# Autodesk Inventor assembly: Caster
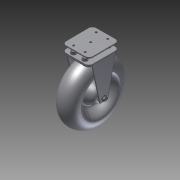
[picture p0: Inventor's stored thumbnail of the model, 180x180]
Saved by Autodesk Inventor 2012 (Build 160160000, 160)
## iProperties
Created: 2011-10-20
Part Number: Caster
Document SubType Name: Assembly
Designer: robotics
Author: robotics
## Documents named in this file (11)
- C:\Users\Tushar\Dropbox\CAD Inventor\Preseason Projects\Cart Competition Cart\Team 2374\Caster.iam
- C:\Users\Tushar\Dropbox\CAD Inventor\Preseason Projects\Cart Competition Cart\Team 2374\Caster2.ipt
- C:\Users\Tushar\Dropbox\CAD Inventor\Preseason Projects\Cart Competition Cart\Team 2374\Wheel.ipt
- C:\Users\Tushar\Dropbox\CAD Inventor\Preseason Projects\Cart Competition Cart\Team 2374\Spacer - .5 x .25.ipt
- C:\Users\Tushar\Dropbox\CAD Inventor\Preseason Projects\Cart Competition Cart\Team 2374\Caster\Design Accelerator\Bolted Connection1.iam
- C:\Users\Tushar\Dropbox\CAD Inventor\Preseason Projects\Cart Competition Cart\Team 2374\Rotation Base.ipt
- C:\Users\Tushar\Dropbox\CAD Inventor\Preseason Projects\Cart Competition Cart\Team 2374\Rotation Top.ipt
- C:\Users\Tushar\Dropbox\CAD Inventor\Preseason Projects\Cart Competition Cart\Team 2374\Caster\Design Accelerator\Bolted Connection2.iam
- C:\Users\Tushar\Dropbox\CAD Inventor\Preseason Projects\Cart Competition Cart\Team 2374\Caster\Design Accelerator\Bolted Connection3.iam
- C:\Users\Tushar\Dropbox\CAD Inventor\Preseason Projects\Cart Competition Cart\Team 2374\Caster\Design Accelerator\Bolted Connection4.iam
- C:\Users\Tushar\Dropbox\CAD Inventor\Preseason Projects\Cart Competition Cart\Team 2374\Caster\Design Accelerator\Bolted Connection5.iam
## Components (11 placed, 6 different names)
1. Caster2:1 — Mate:1, Mate:2, Mate:3, Mate:4, Mate:5, Mate:6, Mate:7, Flush:1, Mate:12, Flush:2, Mate:23, Mate:24
2. Wheel:1 — Mate:1, Mate:2, Mate:3
3. Spacer - .5 x .25:1 — Mate:4, Mate:5
4. Spacer - .5 x .25:2 — Mate:6, Mate:7
5. Bolted Connection:1 [sub-assembly] — Mate:23, Mate:24
6. Rotation Base:1 — Mate:10, Mate:11, Flush:1, Mate:12, Flush:2, Mate:13, Mate:14, Mate:15, Mate:16, Mate:17, Mate:18, Mate:19, Mate:20
7. Rotation Top:1 — Mate:10, Mate:11
8. Bolted Connection:2 [sub-assembly] — Mate:13, Mate:14
9. Bolted Connection:3 [sub-assembly] — Mate:15, Mate:16
10. Bolted Connection:4 [sub-assembly] — Mate:17, Mate:18
11. Bolted Connection:5 [sub-assembly] — Mate:19, Mate:20
## Relationships (22: Mate 20, Flush 2)
- Mate:1 (6.35 mm): Caster2:1 ↔ Wheel:1
- Mate:2 (111.125 mm): Caster2:1 ↔ Wheel:1
- Mate:3 (-50.8 mm): Caster2:1 ↔ Wheel:1
- Mate:4: Caster2:1 ↔ Spacer - .5 x .25:1
- Mate:5: Caster2:1 ↔ Spacer - .5 x .25:1
- Mate:6: Caster2:1 ↔ Spacer - .5 x .25:2
- Mate:7: Caster2:1 ↔ Spacer - .5 x .25:2
- Mate:10: Rotation Base:1 ↔ Rotation Top:1
- Mate:11: Rotation Base:1 ↔ Rotation Top:1
- Flush:1: Caster2:1 ↔ Rotation Base:1
- Mate:12: Caster2:1 ↔ Rotation Base:1
- Flush:2: Caster2:1 ↔ Rotation Base:1
- Mate:13: Rotation Base:1 ↔ Bolted Connection:2
- Mate:14: Rotation Base:1 ↔ Bolted Connection:2
- Mate:15: Rotation Base:1 ↔ Bolted Connection:3
- Mate:16: Rotation Base:1 ↔ Bolted Connection:3
- Mate:17: Rotation Base:1 ↔ Bolted Connection:4
- Mate:18: Rotation Base:1 ↔ Bolted Connection:4
- Mate:19: Rotation Base:1 ↔ Bolted Connection:5
- Mate:20: Rotation Base:1 ↔ Bolted Connection:5
- Mate:23: Caster2:1 ↔ Bolted Connection:1
- Mate:24: Caster2:1 ↔ Bolted Connection:1
